# Autodesk Inventor assembly: ASY ДМФ 0100 Барабан v2.0
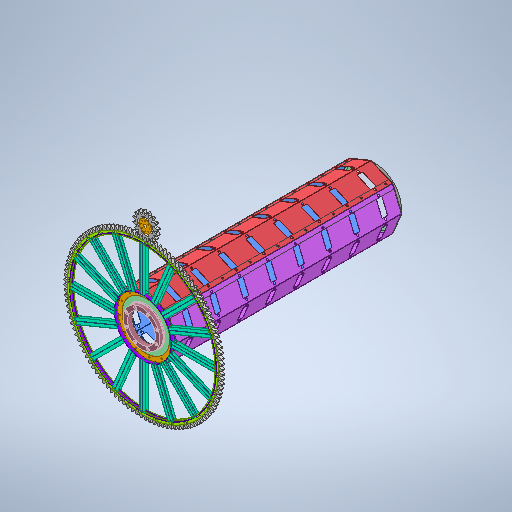
[picture p0: Inventor's stored thumbnail of the model, 512x512]
Saved by Autodesk Inventor 2025 (Build 290162010, 162A)
## iProperties
Created: 2024-04-28
Part Number: ASY ДМФ 0100 Барабан v2.0
Document SubType Name: Assembly
Designer: pokla
Author: pokla
## Documents named in this file (22)
- C:\Users\pokla\Desktop\Эксперимент с колесом\ASY ДМФ 0100 Барабан v2.0.iam
- C:\Users\pokla\Desktop\Эксперимент с колесом\ДМФ 01 21 Барабан торец НОС v2.0.ipt
- C:\Users\pokla\Desktop\Эксперимент с колесом\ДМФ 01 13 Барабан Лист лев брт v2.0.ipt
- C:\Users\pokla\Desktop\Эксперимент с колесом\ДМФ 01 14 Барабан Лист прав брт v2.0.ipt
- C:\Users\pokla\Desktop\Эксперимент с колесом\ДМФ 01 31 Барабан Опорное кольцо НОС v2.0.ipt
- C:\Users\pokla\Desktop\Эксперимент с колесом\ДМФ 01 17 опора крышки v2.0.ipt
- C:\Users\pokla\Desktop\Эксперимент с колесом\ДМФ 000 размеры v2.0.ipt
- C:\Users\pokla\Desktop\Эксперимент с колесом\ДМФ 01 12 Барабан усилитель v2.0.ipt
- C:\Users\pokla\Desktop\Эксперимент с колесом\ASY ДМФ 010 крышка v2.0.iam
- C:\Users\pokla\Desktop\Эксперимент с колесом\ДМФ 01 32 Барабан Опорное кольцо КОРМА v2.0.ipt
- C:\Users\pokla\Desktop\Эксперимент с колесом\ДМФ 01 22 Барабан торец КОРМА v2.0.ipt
- C:\Users\pokla\Desktop\Эксперимент с колесом\ASY фильтр пакет v2.0.iam
- C:\Users\pokla\Desktop\Эксперимент с колесом\ДМФ 01 21 Барабан торец НОС.ipt
- C:\Users\pokla\Desktop\Эксперимент с колесом\DMF2.0 01 42 Gear way 2.ipt
- C:\Users\pokla\Desktop\Эксперимент с колесом\DMF2.0 01 43 Gear rim 3.ipt
- C:\Users\pokla\Desktop\Эксперимент с колесом\DMF2.0 01 44 Gear rim 4.ipt
- C:\Users\pokla\Desktop\Эксперимент с колесом\DMF2.0 01 45 Gear ring 5.ipt
- C:\Users\pokla\Desktop\Эксперимент с колесом\DMF2.0 01 46 Gear axis wheel 6.ipt
- C:\Users\pokla\Desktop\Эксперимент с колесом\ДМФ 01 13 Барабан усилитель v2.0.ipt
- C:\Users\pokla\Desktop\Эксперимент с колесом\small gear.ipt
- C:\Users\pokla\Desktop\Эксперимент с колесом\flange small gear.ipt
- C:\Users\pokla\Desktop\Эксперимент с колесом\sector big gear 2.0.ipt
## Components (110 placed, 21 different names)
1. ДМФ 000 размеры v2.0:1 — Rigid:30
2. ДМФ 01 21 Барабан торец НОС v2.0:2 — Mate:15, Flush:8, Flush:9, Flush:10, Flush:11, Mate:16, Mate:17, Mate:19, Mate:21, Flush:15, Flush:16, Flush:17, Mate:23, Rigid:27, Rigid:29, Rigid:30, Rigid:34
3. ДМФ 01 31 Барабан Опорное кольцо НОС v2.0:1 — Rigid:29
4. ДМФ 01 32 Барабан Опорное кольцо КОРМА v2.0:1 — Rigid:20
5. ДМФ 01 22 Барабан торец КОРМА v2.0:1 — Flush:12, Flush:13, Mate:18, Rigid:20
6. ДМФ 01 13 Барабан Лист лев брт v2.0:1 — Flush:10, Flush:11, Mate:16, Flush:13, Mate:18, Mate:20, Mate:29
7. ДМФ 01 14 Барабан Лист прав брт v2.0:1 — Flush:8, Flush:9, Mate:17, Flush:12, Mate:22, Mate:28
8. ДМФ 01 17 опора крышки v2.0:1 — Mate:21, Flush:15, Mate:22
9. ДМФ 01 17 опора крышки v2.0:2 — Mate:19, Mate:20, Mate:27
10. ASY ДМФ 010 крышка v2.0:1 [sub-assembly] — Flush:16, Flush:17, Mate:23, Mate:27
11. ДМФ 01 29 Барабан сборочный лист:1 — Mate:28, Mate:29
12. DMF2.0 01 45 Gear ring 5:1 — Rigid:21, Rigid:22, Rigid:23, Rigid:27, Rigid:31
13. DMF2.0 01 46 Gear axis wheel 6:1 — Rigid:31
14. small gear:1 — Rigid:33
15. flange small gear:1 — Rigid:33
16. ASY фильтр пакет v2.0:1 [sub-assembly] — Mate:24, Mate:25
17. ASY фильтр пакет v2.0:2 [sub-assembly]
18. ASY фильтр пакет v2.0:3 [sub-assembly]
19. ASY фильтр пакет v2.0:4 [sub-assembly]
20. ASY фильтр пакет v2.0:5 [sub-assembly]
21. ASY фильтр пакет v2.0:6 [sub-assembly]
22. ASY фильтр пакет v2.0:7 [sub-assembly]
23. ASY фильтр пакет v2.0:8 [sub-assembly]
24. DMF2.0 01 43 Gear rim 3:2 — Rigid:24
25. DMF2.0 01 43 Gear rim 3:1 — Rigid:23, Rigid:24
26. DMF2.0 01 43 Gear rim 3:3
27. DMF2.0 01 43 Gear rim 3:6
28. DMF2.0 01 43 Gear rim 3:4
29. DMF2.0 01 43 Gear rim 3:7
30. DMF2.0 01 43 Gear rim 3:5
31. DMF2.0 01 43 Gear rim 3:8
32. DMF2.0 01 44 Gear rim 4:1 — Rigid:22
33. DMF2.0 01 44 Gear rim 4:2
34. DMF2.0 01 44 Gear rim 4:3
35. ДМФ 01 12 Барабан усилитель v2.0:49 — Mate:30, Tangent:1, Mate:31, Rigid:21, Flush:18, Mate:32, Mate:33
36. DMF2.0 01 42 Gear way 2:1 — Mate:30, Tangent:1, Mate:31
37. ДМФ 01 13 Барабан усилитель v2.0:1 — Flush:18, Mate:32, Mate:33
38. ДМФ 01 12 Барабан усилитель v2.0:50
39. DMF2.0 01 42 Gear way 2:2
40. ДМФ 01 13 Барабан усилитель v2.0:2
41. ДМФ 01 12 Барабан усилитель v2.0:51
42. DMF2.0 01 42 Gear way 2:3
43. ДМФ 01 13 Барабан усилитель v2.0:3
44. ДМФ 01 12 Барабан усилитель v2.0:52
45. DMF2.0 01 42 Gear way 2:4
46. ДМФ 01 13 Барабан усилитель v2.0:4
47. ДМФ 01 12 Барабан усилитель v2.0:53
48. DMF2.0 01 42 Gear way 2:5
49. ДМФ 01 13 Барабан усилитель v2.0:5
50. ДМФ 01 12 Барабан усилитель v2.0:54
51. DMF2.0 01 42 Gear way 2:6
52. ДМФ 01 13 Барабан усилитель v2.0:6
53. ДМФ 01 12 Барабан усилитель v2.0:55
54. DMF2.0 01 42 Gear way 2:7
55. ДМФ 01 13 Барабан усилитель v2.0:7
56. ДМФ 01 12 Барабан усилитель v2.0:56
57. DMF2.0 01 42 Gear way 2:8
58. ДМФ 01 13 Барабан усилитель v2.0:8
59. ДМФ 01 12 Барабан усилитель v2.0:57
60. DMF2.0 01 42 Gear way 2:9
61. ДМФ 01 13 Барабан усилитель v2.0:9
62. ДМФ 01 12 Барабан усилитель v2.0:58
63. DMF2.0 01 42 Gear way 2:10
64. ДМФ 01 13 Барабан усилитель v2.0:10
65. ДМФ 01 12 Барабан усилитель v2.0:59
66. DMF2.0 01 42 Gear way 2:11
67. ДМФ 01 13 Барабан усилитель v2.0:11
68. ДМФ 01 12 Барабан усилитель v2.0:60
69. DMF2.0 01 42 Gear way 2:12
70. ДМФ 01 13 Барабан усилитель v2.0:12
71. ДМФ 01 12 Барабан усилитель v2.0:61
72. DMF2.0 01 42 Gear way 2:13
73. ДМФ 01 13 Барабан усилитель v2.0:13
74. ДМФ 01 12 Барабан усилитель v2.0:62
75. DMF2.0 01 42 Gear way 2:14
76. ДМФ 01 13 Барабан усилитель v2.0:14
77. ДМФ 01 12 Барабан усилитель v2.0:63
78. DMF2.0 01 42 Gear way 2:15
79. ДМФ 01 13 Барабан усилитель v2.0:15
80. ДМФ 01 12 Барабан усилитель v2.0:64
81. DMF2.0 01 42 Gear way 2:16
82. ДМФ 01 13 Барабан усилитель v2.0:16
83. sector big gear 2.0:1 — Rigid:34
84. sector big gear 2.0:2
85. sector big gear 2.0:3
86. sector big gear 2.0:4
87. sector big gear 2.0:5
88. sector big gear 2.0:6
89. sector big gear 2.0:7
90. sector big gear 2.0:8
91. sector big gear 2.0:9
92. sector big gear 2.0:10
93. sector big gear 2.0:11
94. sector big gear 2.0:12
95. sector big gear 2.0:13
96. sector big gear 2.0:14
97. sector big gear 2.0:15
98. sector big gear 2.0:16
99. sector big gear 2.0:17
100. sector big gear 2.0:18
101. sector big gear 2.0:19
102. sector big gear 2.0:20
103. sector big gear 2.0:21
104. sector big gear 2.0:22
105. sector big gear 2.0:23
106. sector big gear 2.0:24
107. sector big gear 2.0:25
108. sector big gear 2.0:26
109. sector big gear 2.0:27
110. sector big gear 2.0:28
## Component patterns: (8 elements, first: ASY фильтр пакет v2.0:1), (4 elements, first: DMF2.0 01 43 Gear rim 3:2 + DMF2.0 01 43 Gear rim 3:1), (3 elements, first: DMF2.0 01 44 Gear rim 4:1), (16 elements, first: ДМФ 01 12 Барабан усилитель v2.0:49 + DMF2.0 01 42 Gear way 2:1 + ДМФ 01 13 Барабан усилитель v2.0:1), (28 elements, first: sector big gear 2.0:1)
## Relationships (40: Mate 18, WeldJoint 11, Flush 10, Tangent 1)
- Mate:15: ДМФ 01 21 Барабан торец НОС v2.0:2
- Flush:8: ДМФ 01 21 Барабан торец НОС v2.0:2 ↔ ДМФ 01 14 Барабан Лист прав брт v2.0:1
- Flush:9: ДМФ 01 21 Барабан торец НОС v2.0:2 ↔ ДМФ 01 14 Барабан Лист прав брт v2.0:1
- Flush:10: ДМФ 01 21 Барабан торец НОС v2.0:2 ↔ ДМФ 01 13 Барабан Лист лев брт v2.0:1
- Flush:11: ДМФ 01 21 Барабан торец НОС v2.0:2 ↔ ДМФ 01 13 Барабан Лист лев брт v2.0:1
- Mate:16: ДМФ 01 21 Барабан торец НОС v2.0:2 ↔ ДМФ 01 13 Барабан Лист лев брт v2.0:1
- Mate:17: ДМФ 01 21 Барабан торец НОС v2.0:2 ↔ ДМФ 01 14 Барабан Лист прав брт v2.0:1
- Flush:12: ДМФ 01 22 Барабан торец КОРМА v2.0:1 ↔ ДМФ 01 14 Барабан Лист прав брт v2.0:1
- Flush:13: ДМФ 01 22 Барабан торец КОРМА v2.0:1 ↔ ДМФ 01 13 Барабан Лист лев брт v2.0:1
- Mate:18: ДМФ 01 22 Барабан торец КОРМА v2.0:1 ↔ ДМФ 01 13 Барабан Лист лев брт v2.0:1
- Mate:19: ДМФ 01 21 Барабан торец НОС v2.0:2 ↔ ДМФ 01 17 опора крышки v2.0:2
- Mate:20: ДМФ 01 13 Барабан Лист лев брт v2.0:1 ↔ ДМФ 01 17 опора крышки v2.0:2
- Mate:21: ДМФ 01 21 Барабан торец НОС v2.0:2 ↔ ДМФ 01 17 опора крышки v2.0:1
- Flush:15 (-2 mm): ДМФ 01 21 Барабан торец НОС v2.0:2 ↔ ДМФ 01 17 опора крышки v2.0:1
- Mate:22: ДМФ 01 14 Барабан Лист прав брт v2.0:1 ↔ ДМФ 01 17 опора крышки v2.0:1
- Flush:16: ДМФ 01 21 Барабан торец НОС v2.0:2 ↔ ASY ДМФ 010 крышка v2.0:1
- Flush:17: ДМФ 01 21 Барабан торец НОС v2.0:2 ↔ ASY ДМФ 010 крышка v2.0:1
- Mate:23: ДМФ 01 21 Барабан торец НОС v2.0:2 ↔ ASY ДМФ 010 крышка v2.0:1
- Mate:24: ASY фильтр пакет v2.0:1
- Mate:25: ASY фильтр пакет v2.0:1
- Mate:27: ДМФ 01 17 опора крышки v2.0:2 ↔ ASY ДМФ 010 крышка v2.0:1
- Mate:28: ДМФ 01 14 Барабан Лист прав брт v2.0:1 ↔ ДМФ 01 29 Барабан сборочный лист:1
- Mate:29: ДМФ 01 13 Барабан Лист лев брт v2.0:1 ↔ ДМФ 01 29 Барабан сборочный лист:1
- Rigid:20 [WeldJoint]: ДМФ 01 32 Барабан Опорное кольцо КОРМА v2.0:1 ↔ ДМФ 01 22 Барабан торец КОРМА v2.0:1
- Mate:30: ДМФ 01 12 Барабан усилитель v2.0:49 ↔ DMF2.0 01 42 Gear way 2:1
- Tangent:1: ДМФ 01 12 Барабан усилитель v2.0:49 ↔ DMF2.0 01 42 Gear way 2:1
- Mate:31: ДМФ 01 12 Барабан усилитель v2.0:49 ↔ DMF2.0 01 42 Gear way 2:1
- Rigid:21 [WeldJoint]: DMF2.0 01 45 Gear ring 5:1 ↔ ДМФ 01 12 Барабан усилитель v2.0:49
- Rigid:22 [WeldJoint]: DMF2.0 01 45 Gear ring 5:1 ↔ DMF2.0 01 44 Gear rim 4:1
- Rigid:23 [WeldJoint]: DMF2.0 01 45 Gear ring 5:1 ↔ DMF2.0 01 43 Gear rim 3:1
- Rigid:24 [WeldJoint] (25 mm): DMF2.0 01 43 Gear rim 3:2 ↔ DMF2.0 01 43 Gear rim 3:1
- Rigid:27 [WeldJoint]: ДМФ 01 21 Барабан торец НОС v2.0:2 ↔ DMF2.0 01 45 Gear ring 5:1
- Rigid:29 [WeldJoint]: ДМФ 01 21 Барабан торец НОС v2.0:2 ↔ ДМФ 01 31 Барабан Опорное кольцо НОС v2.0:1
- Rigid:30 [WeldJoint]: ДМФ 000 размеры v2.0:1 ↔ ДМФ 01 21 Барабан торец НОС v2.0:2
- Rigid:31 [WeldJoint]: DMF2.0 01 45 Gear ring 5:1 ↔ DMF2.0 01 46 Gear axis wheel 6:1
- Flush:18: ДМФ 01 12 Барабан усилитель v2.0:49 ↔ ДМФ 01 13 Барабан усилитель v2.0:1
- Mate:32 (2 mm): ДМФ 01 12 Барабан усилитель v2.0:49 ↔ ДМФ 01 13 Барабан усилитель v2.0:1
- Mate:33 (27 mm): ДМФ 01 12 Барабан усилитель v2.0:49 ↔ ДМФ 01 13 Барабан усилитель v2.0:1
- Rigid:33 [WeldJoint]: small gear:1 ↔ flange small gear:1
- Rigid:34 [WeldJoint] (2.5 mm): ДМФ 01 21 Барабан торец НОС v2.0:2 ↔ sector big gear 2.0:1
